# Autodesk Inventor assembly: ShooterAssembly_NERDS
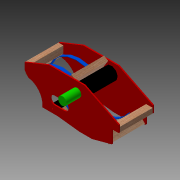
[picture p0: Inventor's stored thumbnail of the model, 180x180]
Saved by Autodesk Inventor 2014 (Build 180170000, 170)
## iProperties
Created: 2016-01-30
Part Number: ShooterAssembly_NERDS
Document SubType Name: Assembly
Designer: bermudezr
Author: bermudezr
## Documents named in this file (13)
- C:\Users\choices.CTE\Documents\Nerds_1726\Models\2015-2016\Assemblies\Robot\Shooter.iam
- C:\Users\choices.CTE\Documents\Nerds_1726\Models\2015-2016\Parts\Robot\Shooter\ShooterMountLeft.ipt
- C:\Users\choices.CTE\Documents\Nerds_1726\Models\2015-2016\Parts\Robot\Shooter\ShooterMountRight.ipt
- C:\Users\choices.CTE\Documents\Nerds_1726\Models\2015-2016\Parts\Robot\Shooter\ShootingMotor.ipt
- C:\Users\choices.CTE\Documents\Nerds_1726\Models\2015-2016\Parts\Robot\Shooter\LoaderMotor.ipt
- C:\Users\choices.CTE\Documents\Nerds_1726\Models\2015-2016\Parts\Robot\Shooter\LoadingRail.ipt
- C:\Users\choices.CTE\Documents\Nerds_1726\Models\2015-2016\Parts\Robot\Shooter\ShootingRail.ipt
- C:\Users\choices.CTE\Documents\Nerds_1726\Models\2015-2016\Parts\Robot\Shooter\SmallMotor.ipt
- C:\Users\choices.CTE\Documents\Nerds_1726\Models\2015-2016\Parts\Robot\Chassis\DriveMotor.ipt
- C:\Users\choices.CTE\Documents\Nerds_1726\Models\2015-2016\Parts\Robot\Shooter\ShieldMount2x4.ipt
- C:\Users\choices.CTE\Documents\Nerds_1726\Models\2015-2016\Parts\Robot\Shooter\ShooterFrontMount.ipt
- C:\Users\choices.CTE\Documents\Nerds_1726\Models\2015-2016\Parts\Robot\Shooter\RailMount2x4.ipt
- C:\Users\choices.CTE\Documents\Nerds_1726\Models\2015-2016\Parts\Robot\Shooter\RailMount1x2.ipt
## Components (15 placed, 12 different names)
1. ShooterMountLeft:1 — Flush:2, Mate:1, Mate:2, Mate:5, Mate:25, Mate:26, Flush:8, Flush:9, Mate:29, Flush:10, Mate:32, Mate:34, Mate:35
2. ShooterMountRight:1 — Flush:2, Mate:1, Mate:3, Mate:12, Insert:2, Flush:6, Flush:7, Mate:31, Flush:10, Mate:33
3. ShootingMotor:1 — Mate:2, Mate:5, Mate:9, Mate:10
4. LoaderMotor:1 — Mate:3, Mate:6, Mate:7, Mate:13, Flush:9, Mate:30
5. LoadingRail:1 — Mate:6, Mate:8, Flush:3, Flush:5, Tangent:9
6. LoadingRail:2 — Mate:7, Mate:8, Flush:5, Mate:12, Tangent:10
7. ShootingRail:1 — Mate:9, Mate:11, Flush:4, Mate:31, Tangent:12, Tangent:13, Tangent:14
8. ShootingRail:2 — Mate:10, Mate:11, Flush:3, Flush:4, Mate:13, Tangent:11
9. SmallMotor:1 — Mate:29, Mate:30
10. DriveMotor:1 — Insert:2
11. ShieldMount2x4:2 — Flush:6, Mate:25, Flush:7
12. ShooterFrontMount:1 — Mate:26, Flush:8, Mate:32
13. RailMount2x4:1 — Mate:33, Tangent:9, Tangent:10
14. RailMount2x4:2 — Tangent:11, Mate:34, Tangent:12
15. RailMount1x2:1 — Mate:35, Tangent:13, Tangent:14
## Relationships (37: Mate 21, Flush 9, Tangent 6, Insert 1)
- Flush:2: ShooterMountLeft:1 ↔ ShooterMountRight:1
- Mate:1 (254 mm): ShooterMountLeft:1 ↔ ShooterMountRight:1
- Mate:2: ShooterMountLeft:1 ↔ ShootingMotor:1
- Mate:3: ShooterMountRight:1 ↔ LoaderMotor:1
- Mate:5: ShooterMountLeft:1 ↔ ShootingMotor:1
- Mate:6: LoaderMotor:1 ↔ LoadingRail:1
- Mate:7: LoaderMotor:1 ↔ LoadingRail:2
- Mate:8 (101.6 mm): LoadingRail:1 ↔ LoadingRail:2
- Mate:9: ShootingMotor:1 ↔ ShootingRail:1
- Mate:10: ShootingMotor:1 ↔ ShootingRail:2
- Mate:11 (101.6 mm): ShootingRail:1 ↔ ShootingRail:2
- Flush:3: LoadingRail:1 ↔ ShootingRail:2
- Flush:4: ShootingRail:1 ↔ ShootingRail:2
- Flush:5: LoadingRail:1 ↔ LoadingRail:2
- Mate:12: ShooterMountRight:1 ↔ LoadingRail:2
- Mate:13 (38.1 mm): LoaderMotor:1 ↔ ShootingRail:2
- Insert:2: ShooterMountRight:1 ↔ DriveMotor:1
- Flush:6: ShooterMountRight:1 ↔ ShieldMount2x4:2
- Mate:25: ShooterMountLeft:1 ↔ ShieldMount2x4:2
- Flush:7: ShooterMountRight:1 ↔ ShieldMount2x4:2
- Mate:26: ShooterMountLeft:1 ↔ ShooterFrontMount:1
- Flush:8: ShooterMountLeft:1 ↔ ShooterFrontMount:1
- Flush:9: ShooterMountLeft:1 ↔ LoaderMotor:1
- Mate:29: ShooterMountLeft:1 ↔ SmallMotor:1
- Mate:30: LoaderMotor:1 ↔ SmallMotor:1
- Mate:31 (50.8 mm): ShooterMountRight:1 ↔ ShootingRail:1
- Flush:10: ShooterMountLeft:1 ↔ ShooterMountRight:1
- Mate:32: ShooterMountLeft:1 ↔ ShooterFrontMount:1
- Mate:33: ShooterMountRight:1 ↔ RailMount2x4:1
- Tangent:9: LoadingRail:1 ↔ RailMount2x4:1
- Tangent:10: LoadingRail:2 ↔ RailMount2x4:1
- Tangent:11: ShootingRail:2 ↔ RailMount2x4:2
- Mate:34: ShooterMountLeft:1 ↔ RailMount2x4:2
- Tangent:12: ShootingRail:1 ↔ RailMount2x4:2
- Mate:35: ShooterMountLeft:1 ↔ RailMount1x2:1
- Tangent:13: ShootingRail:1 ↔ RailMount1x2:1
- Tangent:14: ShootingRail:1 ↔ RailMount1x2:1
